# Autodesk Inventor assembly: whole_setup
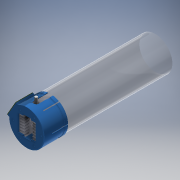
[picture p0: Inventor's stored thumbnail of the model, 180x180]
Saved by Autodesk Inventor 2016 (Build 200138000, 138)
## iProperties
Created: 2016-04-07
Part Number: whole_setup
Document SubType Name: Assembly
Designer: 3DPrinterUser
Author: 3DPrinterUser
## Documents named in this file (9)
- X:\Projekte Bastli\BarBot\Conception\Mechanical\Ice_Dispenser\crusher\whole_setup.iam
- X:\Projekte Bastli\BarBot\Conception\Mechanical\Ice_Dispenser\crusher\pipe_insertv2.ipt
- X:\Projekte Bastli\BarBot\Conception\Mechanical\Ice_Dispenser\crusher\pipe_closure.ipt
- X:\Projekte Bastli\BarBot\Conception\Mechanical\Ice_Dispenser\crusher\axis.ipt
- X:\Projekte Bastli\BarBot\Conception\Mechanical\Ice_Dispenser\crusher\Mutter.ipt
- X:\Projekte Bastli\BarBot\Conception\Mechanical\Ice_Dispenser\crusher\Crusher_Board.ipt
- X:\Projekte Bastli\BarBot\Conception\Mechanical\Ice_Dispenser\crusher\Nut_Normal.ipt
- X:\Projekte Bastli\BarBot\Conception\Mechanical\Ice_Dispenser\crusher\crusher_claw.ipt
- X:\Projekte Bastli\BarBot\Conception\Mechanical\Ice_Dispenser\crusher\Crusher_Tube.ipt
## Components (22 placed, 8 different names)
1. pipe_insertv2:1 — Flush:1, Flush:2, Rotational:1, Rotational:2
2. pipe_closure:1 — Flush:1, Flush:3, Flush:4, Rigid:12
3. axis:1 — Flush:2, Rigid:1
4. Mutter:1 — Rotational:1
5. Mutter:2 — Rotational:2
6. Crusher_Board:1 — Flush:3, Flush:4
7. Nut_Normal:1 — Rigid:2, Rigid:3
8. Mutter:3 — Rotational:5
9. crusher_claw:1 — Rigid:1, Rigid:2, Rotational:6
10. crusher_claw:2 — Rigid:3, Rotational:3
11. Nut_Normal:2 — Rotational:3, Rigid:4
12. crusher_claw:3 — Rigid:4, Rotational:4
13. Nut_Normal:3 — Rotational:4, Rigid:5
14. crusher_claw:4 — Rigid:5, Rotational:5
15. Nut_Normal:4 — Rotational:6, Rotational:7
16. crusher_claw:5 — Rotational:7, Rotational:8
17. Nut_Normal:5 — Rotational:8, Rigid:6
18. crusher_claw:6 — Rigid:6, Rotational:9
19. Mutter:4 — Rotational:10
20. Nut_Normal:6 — Rotational:9, Rigid:7
21. crusher_claw:7 — Rigid:7, Rotational:10
22. Crusher_Tube:1 — Rigid:12
## Relationships (22: RevoluteJoint 10, WeldJoint 8, Flush 4)
- Flush:1: pipe_insertv2:1 ↔ pipe_closure:1
- Flush:2: pipe_insertv2:1 ↔ axis:1
- Rotational:1 [RevoluteJoint]: pipe_insertv2:1 ↔ Mutter:1
- Rotational:2 [RevoluteJoint]: pipe_insertv2:1 ↔ Mutter:2
- Flush:3: pipe_closure:1 ↔ Crusher_Board:1
- Flush:4: pipe_closure:1 ↔ Crusher_Board:1
- Rigid:1 [WeldJoint]: axis:1 ↔ crusher_claw:1
- Rigid:2 [WeldJoint]: Nut_Normal:1 ↔ crusher_claw:1
- Rigid:3 [WeldJoint]: Nut_Normal:1 ↔ crusher_claw:2
- Rotational:3 [RevoluteJoint]: crusher_claw:2 ↔ Nut_Normal:2
- Rigid:4 [WeldJoint]: Nut_Normal:2 ↔ crusher_claw:3
- Rotational:4 [RevoluteJoint]: crusher_claw:3 ↔ Nut_Normal:3
- Rigid:5 [WeldJoint]: Nut_Normal:3 ↔ crusher_claw:4
- Rotational:5 [RevoluteJoint]: Mutter:3 ↔ crusher_claw:4
- Rotational:6 [RevoluteJoint]: crusher_claw:1 ↔ Nut_Normal:4
- Rotational:7 [RevoluteJoint]: Nut_Normal:4 ↔ crusher_claw:5
- Rotational:8 [RevoluteJoint]: crusher_claw:5 ↔ Nut_Normal:5
- Rigid:6 [WeldJoint]: Nut_Normal:5 ↔ crusher_claw:6
- Rotational:9 [RevoluteJoint]: crusher_claw:6 ↔ Nut_Normal:6
- Rigid:7 [WeldJoint]: Nut_Normal:6 ↔ crusher_claw:7
- Rotational:10 [RevoluteJoint]: Mutter:4 ↔ crusher_claw:7
- Rigid:12 [WeldJoint]: pipe_closure:1 ↔ Crusher_Tube:1
